# Autodesk Inventor assembly: Assembly_Eyepiece_Folded
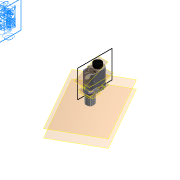
[picture p0: Inventor's stored thumbnail of the model, 180x180]
Saved by Autodesk Inventor 2019 (Build 230136000, 136)
## iProperties
Created: 2019-11-14
Part Number: Assembly_Eyepiece_Folded
Document SubType Name: Assembly
Designer: diederichbenedict
Author: diederichbenedict
## Documents named in this file (6)
- C:\Users\diederichbenedict\Dropbox\Dokumente\Promotion\PROJECTS\STORMoChip\INVENTOR\Nanoscopy-on-a-cheap\Assembly_Eyepiece_Folded.iam
- C:\Users\diederichbenedict\Dropbox\Dokumente\Promotion\PROJECTS\STORMoChip\INVENTOR\Nanoscopy-on-a-cheap\00_Eyepiece_20x_WF.ipt
- C:\Users\diederichbenedict\Dropbox\Dokumente\Promotion\PROJECTS\STORMoChip\INVENTOR\Nanoscopy-on-a-cheap\00_Microscope_Objective.ipt
- C:\Users\diederichbenedict\Dropbox\Dokumente\Promotion\PROJECTS\STORMoChip\INVENTOR\Nanoscopy-on-a-cheap\PF10-03-P01-Step.ipt
- C:\Users\diederichbenedict\Dropbox\Dokumente\Promotion\PROJECTS\STORMoChip\INVENTOR\Nanoscopy-on-a-cheap\00_Beam_Ocular_Detectoin.ipt
- C:\Users\diederichbenedict\Dropbox\Dokumente\Promotion\PROJECTS\STORMoChip\INVENTOR\Nanoscopy-on-a-cheap\cellSTORM_objective_tube_folded_mirror_v0.ipt
## Components (6 placed, 5 different names)
1. 00_Eyepiece_20x_WF:1 — Insert:5
2. 00_Microscope_Objective:1 — Insert:2
3. PF10-03-P01-Step:1 — Insert:3
4. PF10-03-P01-Step:2 — Insert:4
5. 00_Beam_Ocular_Detectoin:1 — Insert:2, Insert:3, Insert:4, Insert:5
6. cellSTORM_objective_tube_folded_mirror_v0:1
## Relationships (4: Insert 4)
- Insert:2: 00_Microscope_Objective:1 ↔ 00_Beam_Ocular_Detectoin:1
- Insert:3: PF10-03-P01-Step:1 ↔ 00_Beam_Ocular_Detectoin:1
- Insert:4: PF10-03-P01-Step:2 ↔ 00_Beam_Ocular_Detectoin:1
- Insert:5: 00_Eyepiece_20x_WF:1 ↔ 00_Beam_Ocular_Detectoin:1
